# Autodesk Inventor assembly: Arm_MiniLink_Shim_i_8
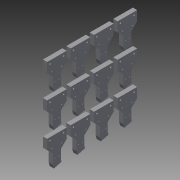
[picture p0: Inventor's stored thumbnail of the model, 180x180]
Saved by Autodesk Inventor 2013 (Build 170138000, 138)
## iProperties
Created: 2014-05-17
Part Number: Arm_MiniLink_Shim_i_8
Document SubType Name: Assembly
Designer: andou
Author: andou
## Documents named in this file (2)
- C:\Users\andou\Documents\Inventor\RoboticsProject\project_4\Robot\Arm\Arm_MiniLink_Shim_i_8.iam
- C:\Users\andou\Documents\Inventor\RoboticsProject\project_4\Robot\Arm\Arm_MiniLink_Shim_i.ipt
## Components (12 placed, 1 different names)
1. Arm_MiniLink_Shim_i:1
2. Arm_MiniLink_Shim_i:2
3. Arm_MiniLink_Shim_i:3
4. Arm_MiniLink_Shim_i:4
5. Arm_MiniLink_Shim_i:5
6. Arm_MiniLink_Shim_i:6
7. Arm_MiniLink_Shim_i:7
8. Arm_MiniLink_Shim_i:8
9. Arm_MiniLink_Shim_i:9
10. Arm_MiniLink_Shim_i:10
11. Arm_MiniLink_Shim_i:11
12. Arm_MiniLink_Shim_i:12
## Component patterns: (12 elements, first: Arm_MiniLink_Shim_i:1)
